# Autodesk Inventor assembly: Assembly
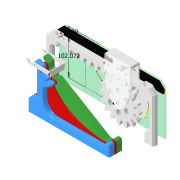
[picture p0: Inventor's stored thumbnail of the model, 180x180]
Saved by Autodesk Inventor 2020 (Build 240168000, 168)
## iProperties
Created: 2021-07-09
Part Number: Assembly
Document SubType Name: Assembly
Designer: Aidan Lee
Author: Aidan Lee
## Documents named in this file (4)
- C:\Users\hobly\Dropbox\Aidan Lee\Mechanics_Walk\Brachistochrone-v2\BrachistochroneFullAssembly.iam
- C:\Users\hobly\Dropbox\Aidan Lee\Mechanics_Walk\Brachistochrone-v2\CycloidDrawer.iam
- C:\Users\hobly\Dropbox\Aidan Lee\Mechanics_Walk\Brachistochrone-v2\BrachistochroneCurvedPaths.iam
- C:\Users\hobly\Dropbox\Aidan Lee\Mechanics_Walk\Brachistochrone-v2\platform.ipt
## Components (3 placed, 3 different names)
1. CycloidDrawer:1 [sub-assembly] — Flush:1, Flush:2, Mate:1, Mate:3, Flush:3, Mate:5, Mate:6
2. BrachistochroneCurvedPaths:1 [sub-assembly] — Flush:1, Flush:2, Mate:1, Mate:2, Mate:4
3. platform:1 — Mate:4, Mate:5, Mate:6
## Relationships (9: Mate 6, Flush 3)
- Flush:1: CycloidDrawer:1 ↔ BrachistochroneCurvedPaths:1
- Flush:2 (-36.567 mm): CycloidDrawer:1 ↔ BrachistochroneCurvedPaths:1
- Mate:1 (50 mm): CycloidDrawer:1 ↔ BrachistochroneCurvedPaths:1
- Mate:2: BrachistochroneCurvedPaths:1
- Mate:3 (25 mm): CycloidDrawer:1
- Flush:3: CycloidDrawer:1
- Mate:4: BrachistochroneCurvedPaths:1 ↔ platform:1
- Mate:5: CycloidDrawer:1 ↔ platform:1
- Mate:6: CycloidDrawer:1 ↔ platform:1
